# Autodesk Inventor assembly: cam_holder
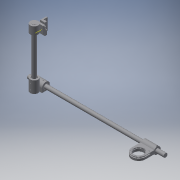
[picture p0: Inventor's stored thumbnail of the model, 180x180]
Saved by Autodesk Inventor 2019 (Build 230136000, 136)
## iProperties
Created: 2024-08-06
Part Number: cam_holder
Material: Generisch
Document SubType Name: Assembly
Designer: nic
Author: nic
## Documents named in this file (7)
- C:\Users\Nicolas Frick\Sync\OneDrive\wtm\nicol_rh8d\atxmega_qenc\inventor\cam_holder.iam
- C:\Users\Nicolas Frick\Sync\OneDrive\wtm\nicol_rh8d\atxmega_qenc\inventor\pipe_700.ipt
- C:\Users\Nicolas Frick\Sync\OneDrive\wtm\nicol_rh8d\atxmega_qenc\inventor\pipe_300.ipt
- C:\Users\Nicolas Frick\Sync\OneDrive\wtm\nicol_rh8d\atxmega_qenc\inventor\cam_holder_wrist_part_aligned.iam
- C:\Users\Nicolas Frick\Sync\OneDrive\wtm\nicol_rh8d\atxmega_qenc\inventor\cam_holder_angle_part_aligned.iam
- C:\Users\Nicolas Frick\Sync\OneDrive\wtm\nicol_rh8d\atxmega_qenc\inventor\cam_holder_end_part_aligned.iam
- C:\Users\Nicolas Frick\Sync\OneDrive\wtm\nicol_rh8d\atxmega_qenc\inventor\cam_holder_hog_part_aligned.iam
## Components (6 placed, 6 different names)
1. pipe_700:1 — Passend:1, Passend:2
2. pipe_300:1 — Passend:5, Passend:6
3. cam_holder_wrist_part_aligned:1 [sub-assembly] — Fluchtend:3, Passend:1, distance_from_hand, angle_from_hand_x, Passend:4, angle_from_hand_z
4. cam_holder_angle_part_aligned:1 [sub-assembly] — Passend:2, distance_from_hand, angle_from_hand_x, Passend:5, distance_from_flange, camera_z_angle
5. cam_holder_end_part_aligned:1 [sub-assembly] — Passend:6, distance_from_flange, camera_z_angle, Passend:8, Passend:9, camera_y_angle
6. cam_holder_hog_part_aligned:1 [sub-assembly] — Passend:8, Passend:9, camera_y_angle
## Relationships (14: Mate 9, Angle 4, Flush 1)
- Fluchtend:3 [Flush]: cam_holder_wrist_part_aligned:1
- Passend:1 [Mate]: pipe_700:1 ↔ cam_holder_wrist_part_aligned:1
- Passend:2 [Mate]: pipe_700:1 ↔ cam_holder_angle_part_aligned:1
- distance_from_hand [Mate] (500 mm): cam_holder_wrist_part_aligned:1 ↔ cam_holder_angle_part_aligned:1
- angle_from_hand_x (0 deg): cam_holder_wrist_part_aligned:1 ↔ cam_holder_angle_part_aligned:1
- Passend:4 [Mate]: cam_holder_wrist_part_aligned:1
- angle_from_hand_z (0 deg): cam_holder_wrist_part_aligned:1
- Passend:5 [Mate]: pipe_300:1 ↔ cam_holder_angle_part_aligned:1
- Passend:6 [Mate]: pipe_300:1 ↔ cam_holder_end_part_aligned:1
- distance_from_flange [Mate] (200 mm): cam_holder_angle_part_aligned:1 ↔ cam_holder_end_part_aligned:1
- camera_z_angle [Angle] (0 deg): cam_holder_angle_part_aligned:1 ↔ cam_holder_end_part_aligned:1
- Passend:8 [Mate]: cam_holder_end_part_aligned:1 ↔ cam_holder_hog_part_aligned:1
- Passend:9 [Mate]: cam_holder_end_part_aligned:1 ↔ cam_holder_hog_part_aligned:1
- camera_y_angle [Angle] (0 deg): cam_holder_end_part_aligned:1 ↔ cam_holder_hog_part_aligned:1
